# Autodesk Inventor assembly: Ankle_independent_pitch
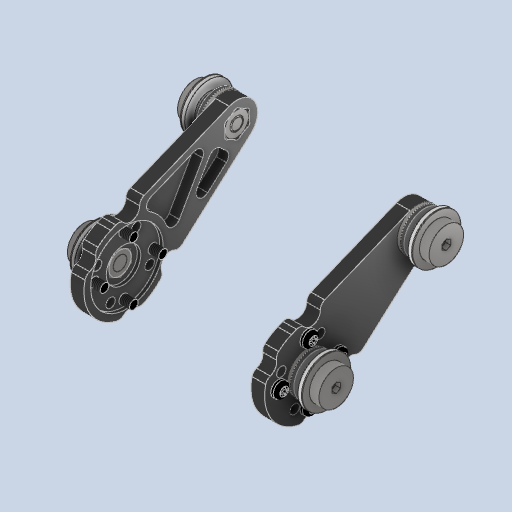
[picture p0: Inventor's stored thumbnail of the model, 512x512]
Saved by Autodesk Inventor 2022.5 (Build 265521000, 521)
## iProperties
Created: 2023-09-22
Part Number: Ankle_independent_pitch
Document SubType Name: Assembly
Designer: Masato Kubotera
Author: Masato Kubotera
## Documents named in this file (3)
- C:\Users\Masato\Documents\Inventor\SUSTAINA-OP\ModelingFiles\LowerBody\Ankle\Ankle_independent_pitch.iam
- C:\Users\Masato\Documents\Inventor\SUSTAINA-OP\ModelingFiles\LowerBody\Ankle\Ankle_side_pitch.iam
- C:\Users\Masato\Documents\Inventor\SUSTAINA-OP\ModelingFiles\COTS\Screw\F-2606EB.ipt
## Components (10 placed, 2 different names)
1. Ankle_side_pitch:1 [sub-assembly] — 挿入:1, 挿入:2, 挿入:3, 挿入:4, フラッシュ:1, フラッシュ:2, フラッシュ:3, フラッシュ:4
2. Ankle_side_pitch:2 [sub-assembly] — 挿入:5, 挿入:6, 挿入:7, 挿入:8, メイト:1, メイト:2, フラッシュ:4
3. F-2606EB:1 — 挿入:1
4. F-2606EB:2 — 挿入:2
5. F-2606EB:3 — 挿入:3
6. F-2606EB:4 — 挿入:4
7. F-2606EB:5 — 挿入:5
8. F-2606EB:6 — 挿入:6
9. F-2606EB:7 — 挿入:7
10. F-2606EB:8 — 挿入:8
## Relationships (14: Insert 8, Flush 4, Mate 2)
- 挿入:1 [Insert]: Ankle_side_pitch:1 ↔ F-2606EB:1
- 挿入:2 [Insert]: Ankle_side_pitch:1 ↔ F-2606EB:2
- 挿入:3 [Insert]: Ankle_side_pitch:1 ↔ F-2606EB:3
- 挿入:4 [Insert]: Ankle_side_pitch:1 ↔ F-2606EB:4
- 挿入:5 [Insert]: Ankle_side_pitch:2 ↔ F-2606EB:5
- 挿入:6 [Insert]: Ankle_side_pitch:2 ↔ F-2606EB:6
- 挿入:7 [Insert]: Ankle_side_pitch:2 ↔ F-2606EB:7
- 挿入:8 [Insert]: Ankle_side_pitch:2 ↔ F-2606EB:8
- フラッシュ:1 [Flush]: Ankle_side_pitch:1
- フラッシュ:2 [Flush]: Ankle_side_pitch:1
- フラッシュ:3 [Flush]: Ankle_side_pitch:1
- メイト:1 [Mate]: Ankle_side_pitch:2
- メイト:2 [Mate]: Ankle_side_pitch:2
- フラッシュ:4 [Flush]: Ankle_side_pitch:1 ↔ Ankle_side_pitch:2
